# Autodesk Inventor assembly: 79. Головка заднего хода в сборе
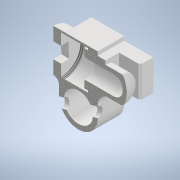
[picture p0: Inventor's stored thumbnail of the model, 180x180]
Saved by Autodesk Inventor 2021 (Build 250183000, 183)
## iProperties
Created: 2021-04-02
Part Number: 79. Головка заднего хода в сборе
Document SubType Name: Assembly
Designer: Данил
Author: Данил
## Documents named in this file (4)
- C:\Users\Данил\Desktop\Коробка передач\Детали\79. Головка заднего хода в сборе.iam
- C:\Users\Данил\Desktop\Коробка передач\Детали\411. Головка штока заднего хода.ipt
- C:\Users\Данил\Desktop\Коробка передач\Детали\79. Предохранитель заднего хода.ipt
- C:\Users\Данил\Desktop\Коробка передач\Детали\80. Стопор предохранителя.ipt
## Components (3 placed, 3 different names)
1. 411. Головка штока заднего хода:1 — Совмещение:1, Заподлицо:1, Совмещение:2, Совмещение:3
2. 79. Предохранитель заднего хода:1 — Совмещение:2, Совмещение:3
3. 80. Стопор предохранителя:1 — Совмещение:1, Заподлицо:1
## Relationships (4: Mate 3, Flush 1)
- Совмещение:1 [Mate]: 411. Головка штока заднего хода:1 ↔ 80. Стопор предохранителя:1
- Заподлицо:1 [Flush]: 411. Головка штока заднего хода:1 ↔ 80. Стопор предохранителя:1
- Совмещение:2 [Mate]: 411. Головка штока заднего хода:1 ↔ 79. Предохранитель заднего хода:1
- Совмещение:3 [Mate]: 411. Головка штока заднего хода:1 ↔ 79. Предохранитель заднего хода:1
